# Autodesk Inventor assembly: Gripper
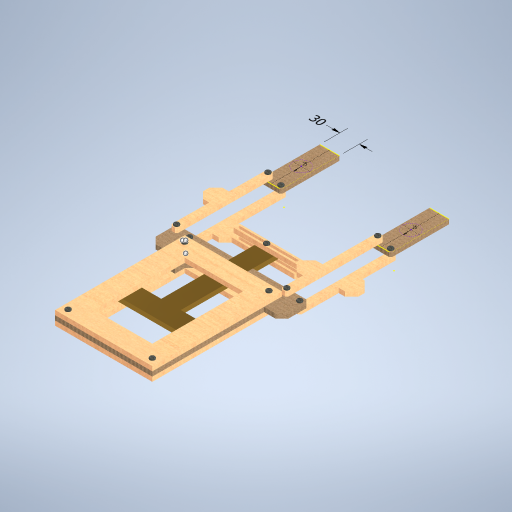
[picture p0: Inventor's stored thumbnail of the model, 512x512]
Saved by Autodesk Inventor 2023.1 (Build 271208000, 208)
## iProperties
Created: 2022-10-28
Part Number: Gripper
Document SubType Name: Assembly
Designer: Daniel Peña
Author: Daniel Peña
## Documents named in this file (9)
- E:\Daniel DiscoA\Documents\UNAL\ProyectoRobotica\CAD\Gripper.iam
- E:\Daniel DiscoA\Documents\UNAL\ProyectoRobotica\CAD\Base.ipt
- E:\Daniel DiscoA\Documents\UNAL\ProyectoRobotica\CAD\Marco.ipt
- E:\Daniel DiscoA\Documents\UNAL\ProyectoRobotica\CAD\Piston.ipt
- E:\Daniel DiscoA\Documents\UNAL\ProyectoRobotica\CAD\Dedo.ipt
- E:\Daniel DiscoA\Documents\UNAL\ProyectoRobotica\CAD\Lever.ipt
- E:\Daniel DiscoA\Documents\UNAL\ProyectoRobotica\CAD\tLever.ipt
- E:\Daniel DiscoA\Documents\Inventor\Content Center Files\R2023\en-US\ISO 7045  H\ISO 7045 - M4 x 25_ - 4.8 - H - ISO.ipt
- E:\Daniel DiscoA\Documents\Inventor\Content Center Files\R2023\en-US\ISO 7045  H\ISO 7045 - M4 x 16_ - 4.8 - H - ISO.ipt
## Components (23 placed, 8 different names)
1. Base:1 — Flush:1, Mate:2
2. Marco:1 — Flush:1, Flush:4, Mate:1, Rotational:1, Rotational:7, Mate:3, Mate:4, Rotational:11, Rotational:12, Mate:25, Mate:26, Mate:29, Mate:30
3. Piston:1 — Mate:2, Mate:3, Mate:4, Mate:13
4. Base:2 — Flush:4, Mate:1, Mate:5, Mate:6, Mate:7, Mate:8, Mate:9, Mate:10, Mate:11, Mate:12
5. Dedo:1 — Rotational:2, Rotational:14, Mate:21, Mate:22
6. Dedo:2 — Rotational:10, Rotational:13, Mate:17, Mate:18
7. Lever:1 — Rotational:1, Rotational:2, Mate:19, Mate:20, Mate:23, Mate:24
8. Lever:2 — Rotational:7, Rotational:10
9. tLever:1 — Rotational:12, Rotational:14
10. tLever:2 — Rotational:11, Rotational:13, Mate:14, Mate:15, Mate:16, Mate:27, Mate:28
11. ISO 7045 H M4 x 25 - 4.8 - H:1 — Mate:5, Mate:6
12. ISO 7045 H M4 x 25 - 4.8 - H:2 — Mate:7, Mate:8
13. ISO 7045 H M4 x 25 - 4.8 - H:3 — Mate:9, Mate:10
14. ISO 7045 H M4 x 25 - 4.8 - H:4 — Mate:11, Mate:12
15. ISO 7045 H M4 x 25 - 4.8 - H:5 — Mate:13, Mate:14
16. ISO 7045 H M4 x 16 - 4.8 - H:1 — Mate:15, Mate:16
17. ISO 7045 H M4 x 16 - 4.8 - H:2 — Mate:17, Mate:18
18. ISO 7045 H M4 x 16 - 4.8 - H:3 — Mate:19, Mate:20
19. ISO 7045 H M4 x 16 - 4.8 - H:4 — Mate:21, Mate:22
20. ISO 7045 H M4 x 16 - 4.8 - H:5 — Mate:23, Mate:24
21. ISO 7045 H M4 x 16 - 4.8 - H:6 — Mate:25, Mate:26
22. ISO 7045 H M4 x 16 - 4.8 - H:7 — Mate:27, Mate:28
23. ISO 7045 H M4 x 16 - 4.8 - H:8 — Mate:29, Mate:30
## Relationships (40: Mate 30, RevoluteJoint 8, Flush 2)
- Flush:1: Base:1 ↔ Marco:1
- Flush:4: Marco:1 ↔ Base:2
- Mate:1: Marco:1 ↔ Base:2
- Rotational:1 [RevoluteJoint]: Marco:1 ↔ Lever:1
- Rotational:2 [RevoluteJoint]: Dedo:1 ↔ Lever:1
- Rotational:7 [RevoluteJoint]: Marco:1 ↔ Lever:2
- Rotational:10 [RevoluteJoint]: Dedo:2 ↔ Lever:2
- Mate:2: Base:1 ↔ Piston:1
- Mate:3: Marco:1 ↔ Piston:1
- Mate:4: Marco:1 ↔ Piston:1
- Rotational:11 [RevoluteJoint]: Marco:1 ↔ tLever:2
- Rotational:12 [RevoluteJoint]: Marco:1 ↔ tLever:1
- Rotational:13 [RevoluteJoint]: Dedo:2 ↔ tLever:2
- Rotational:14 [RevoluteJoint]: Dedo:1 ↔ tLever:1
- Mate:5: Base:2 ↔ ISO 7045 H M4 x 25 - 4.8 - H:1
- Mate:6: Base:2 ↔ ISO 7045 H M4 x 25 - 4.8 - H:1
- Mate:7: Base:2 ↔ ISO 7045 H M4 x 25 - 4.8 - H:2
- Mate:8: Base:2 ↔ ISO 7045 H M4 x 25 - 4.8 - H:2
- Mate:9: Base:2 ↔ ISO 7045 H M4 x 25 - 4.8 - H:3
- Mate:10: Base:2 ↔ ISO 7045 H M4 x 25 - 4.8 - H:3
- Mate:11: Base:2 ↔ ISO 7045 H M4 x 25 - 4.8 - H:4
- Mate:12: Base:2 ↔ ISO 7045 H M4 x 25 - 4.8 - H:4
- Mate:13: Piston:1 ↔ ISO 7045 H M4 x 25 - 4.8 - H:5
- Mate:14: tLever:2 ↔ ISO 7045 H M4 x 25 - 4.8 - H:5
- Mate:15: tLever:2 ↔ ISO 7045 H M4 x 16 - 4.8 - H:1
- Mate:16: tLever:2 ↔ ISO 7045 H M4 x 16 - 4.8 - H:1
- Mate:17: Dedo:2 ↔ ISO 7045 H M4 x 16 - 4.8 - H:2
- Mate:18: Dedo:2 ↔ ISO 7045 H M4 x 16 - 4.8 - H:2
- Mate:19: Lever:1 ↔ ISO 7045 H M4 x 16 - 4.8 - H:3
- Mate:20: Lever:1 ↔ ISO 7045 H M4 x 16 - 4.8 - H:3
- Mate:21: Dedo:1 ↔ ISO 7045 H M4 x 16 - 4.8 - H:4
- Mate:22: Dedo:1 ↔ ISO 7045 H M4 x 16 - 4.8 - H:4
- Mate:23: Lever:1 ↔ ISO 7045 H M4 x 16 - 4.8 - H:5
- Mate:24: Lever:1 ↔ ISO 7045 H M4 x 16 - 4.8 - H:5
- Mate:25: Marco:1 ↔ ISO 7045 H M4 x 16 - 4.8 - H:6
- Mate:26: Marco:1 ↔ ISO 7045 H M4 x 16 - 4.8 - H:6
- Mate:27: tLever:2 ↔ ISO 7045 H M4 x 16 - 4.8 - H:7
- Mate:28: tLever:2 ↔ ISO 7045 H M4 x 16 - 4.8 - H:7
- Mate:29: Marco:1 ↔ ISO 7045 H M4 x 16 - 4.8 - H:8
- Mate:30: Marco:1 ↔ ISO 7045 H M4 x 16 - 4.8 - H:8
## Named parameters: hMDF = 7 mm
